# Autodesk Inventor assembly: Rack and Pinion Gearbox Assembly
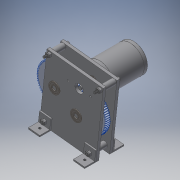
[picture p0: Inventor's stored thumbnail of the model, 180x180]
Saved by Autodesk Inventor 2018 (Build 220112000, 112)
## iProperties
Created: 2019-01-29
Part Number: Rack and Pinion Gearbox Assembly
Document SubType Name: Assembly
Designer: maste
Author: maste
## Documents named in this file (14)
- C:\Users\maste\OneDrive\Documents\GitHub\2019CAD\Drivebase but Calvin is a mad man\Rack and Pinion Gearbox Assembly.iam
- C:\Users\maste\OneDrive\Documents\GitHub\2019CAD\Drivebase but Calvin is a mad man\Rack and Pinion Gearbox Plate.ipt
- C:\Users\maste\OneDrive\Documents\GitHub\2019CAD\Drivebase but Calvin is a mad man\12t_Steel_Spur_Gear_20_DP_CIM_Motor_217-3099.ipt
- C:\Users\maste\OneDrive\Documents\GitHub\2019CAD\Drivebase but Calvin is a mad man\14t_Steel_Spur_Gear_20_DP_3_8_Hex_Bore_217-3100.step.ipt
- C:\Users\maste\OneDrive\Documents\GitHub\2019CAD\Drivebase but Calvin is a mad man\72t_Aluminum_Spur_Gear_20_DP_1_2_Hex_Bore_217-3576.ipt
- C:\Users\maste\OneDrive\Documents\GitHub\2019CAD\Drivebase but Calvin is a mad man\am-3832 375H to 500H Adapter.ipt
- C:\Users\maste\OneDrive\Documents\GitHub\2019CAD\Drivebase but Calvin is a mad man\Mini_CIM_Motor_217-3371.ipt
- C:\Users\maste\OneDrive\Documents\GitHub\2019CAD\Drivebase but Calvin is a mad man\10_25mm_3_8_ThunderHex_ID_x_0_875_OD_x_0_280_WD_Flanged_Bearing_217-5829 (1).ipt
- C:\Users\maste\OneDrive\Documents\GitHub\2019CAD\Drivebase but Calvin is a mad man\92196A272_18-8 STAINLESS STEEL SOCKET HEAD CAP SCREW.ipt
- C:\Users\maste\OneDrive\Documents\GitHub\2019CAD\Drivebase but Calvin is a mad man\Not Tiberculosis TB Hex Shaft.ipt
- C:\Users\maste\OneDrive\Documents\GitHub\2019CAD\Drivebase but Calvin is a mad man\I'm not awake enough to be making churros.ipt
- C:\Users\maste\OneDrive\Documents\GitHub\2019CAD\Drivebase but Calvin is a mad man\L-Bracket L.ipt
- C:\Users\maste\OneDrive\Documents\GitHub\2019CAD\Drivebase but Calvin is a mad man\92196A253_18-8 STAINLESS STEEL SOCKET HEAD CAP SCREW.ipt
- C:\Users\maste\OneDrive\Documents\GitHub\2019CAD\Drivebase but Calvin is a mad man\91831A011_TYPE 18-8 STAINLESS STL NYLON-INSERT LOCKNUT.ipt
## Components (33 placed, 13 different names)
1. Rack and Pinion Gearbox Plate:1 — Mate:1, Mate:2, Mate:3, Mate:6, Mate:7, Mate:8, Mate:9, Mate:10, Mate:11, Mate:12, Mate:13, Mate:20, Flush:3, Flush:4, Flush:8, Mate:48, Mate:49, Flush:9, Mate:50, Mate:51, Mate:52, Mate:53, Mate:56, Mate:57
2. Rack and Pinion Gearbox Plate:2 — Mate:24, Mate:25, Mate:26, Mate:27, Flush:3, Flush:4, Mate:36, Mate:37, Mate:38, Mate:39, Mate:40, Mate:41, Mate:42, Mate:43, Mate:44, Mate:45, Flush:6, Mate:46, Mate:47, Flush:7, Mate:60, Mate:61
3. 12t_Steel_Spur_Gear_20_DP_CIM_Motor_217-3099:1 — Mate:4, Mate:5, Flush:1
4. 14t_Steel_Spur_Gear_20_DP_3_8_Hex_Bore_217-3100.step:1 — Mate:21, Mate:22, Mate:23
5. 72t_Aluminum_Spur_Gear_20_DP_1_2_Hex_Bore_217-3576:1 — Mate:14, Mate:15, Flush:2, Mate:20, Mate:23, Mate:34
6. 72t_Aluminum_Spur_Gear_20_DP_1_2_Hex_Bore_217-3576:2 — Mate:30, Mate:31, Flush:5, Mate:34, Mate:35
7. am-3832 375H to 500H Adapter:1 — Mate:14, Mate:15, Flush:2, Mate:18, Mate:19
8. am-3832 375H to 500H Adapter:2 — Mate:30, Mate:31, Flush:5, Mate:32, Mate:33
9. Mini_CIM_Motor_217-3371:1 — Mate:1, Mate:2, Mate:3, Mate:4, Mate:5, Flush:1
10. 10_25mm_3_8_ThunderHex_ID_x_0_875_OD_x_0_280_WD_Flanged_Bearing_217-5829 (1):1 — Mate:24, Mate:25, Mate:35
11. 10_25mm_3_8_ThunderHex_ID_x_0_875_OD_x_0_280_WD_Flanged_Bearing_217-5829 (1):2 — Mate:26, Mate:27
12. 10_25mm_3_8_ThunderHex_ID_x_0_875_OD_x_0_280_WD_Flanged_Bearing_217-5829 (1):3 — Mate:8, Mate:9, Mate:28, Mate:29
13. 10_25mm_3_8_ThunderHex_ID_x_0_875_OD_x_0_280_WD_Flanged_Bearing_217-5829 (1):4 — Mate:6, Mate:7, Mate:16, Mate:17
14. 92196A272_18-8 STAINLESS STEEL SOCKET HEAD CAP SCREW:1 — Mate:10, Mate:13
15. 92196A272_18-8 STAINLESS STEEL SOCKET HEAD CAP SCREW:2 — Mate:11, Mate:12
16. Not Tiberculosis TB Hex Shaft:1 — Mate:16, Mate:17, Mate:18, Mate:19, Mate:21, Mate:22
17. Not Tiberculosis TB Hex Shaft:2 — Mate:28, Mate:29, Mate:32, Mate:33
18. I'm not awake enough to be making churros:1 — Mate:36, Mate:42
19. I'm not awake enough to be making churros:2 — Mate:38, Mate:43
20. I'm not awake enough to be making churros:3 — Mate:39, Mate:40
21. I'm not awake enough to be making churros:4 — Mate:37, Mate:41
22. L-Bracket L:1 — Flush:9, Mate:50, Mate:51, Mate:55, Mate:58
23. L-Bracket L:2 — Flush:8, Mate:48, Mate:49, Mate:54, Mate:59
24. L-Bracket L:3 — Mate:44, Mate:45, Flush:6, Mate:63
25. L-Bracket L:4 — Mate:46, Mate:47, Flush:7, Mate:62
26. 92196A253_18-8 STAINLESS STEEL SOCKET HEAD CAP SCREW:1 — Mate:54, Mate:59, Mate:65
27. 92196A253_18-8 STAINLESS STEEL SOCKET HEAD CAP SCREW:2 — Mate:55, Mate:58, Mate:64
28. 92196A253_18-8 STAINLESS STEEL SOCKET HEAD CAP SCREW:3 — Mate:52, Mate:56, Mate:67
29. 92196A253_18-8 STAINLESS STEEL SOCKET HEAD CAP SCREW:4 — Mate:53, Mate:57, Mate:66
30. 91831A011_TYPE 18-8 STAINLESS STL NYLON-INSERT LOCKNUT:1 — Mate:62, Mate:64
31. 91831A011_TYPE 18-8 STAINLESS STL NYLON-INSERT LOCKNUT:2 — Mate:63, Mate:65
32. 91831A011_TYPE 18-8 STAINLESS STL NYLON-INSERT LOCKNUT:3 — Mate:60, Mate:67
33. 91831A011_TYPE 18-8 STAINLESS STL NYLON-INSERT LOCKNUT:4 — Mate:61, Mate:66
## Relationships (76: Mate 67, Flush 9)
- Mate:1: Rack and Pinion Gearbox Plate:1 ↔ Mini_CIM_Motor_217-3371:1
- Mate:2: Rack and Pinion Gearbox Plate:1 ↔ Mini_CIM_Motor_217-3371:1
- Mate:3: Rack and Pinion Gearbox Plate:1 ↔ Mini_CIM_Motor_217-3371:1
- Mate:4: 12t_Steel_Spur_Gear_20_DP_CIM_Motor_217-3099:1 ↔ Mini_CIM_Motor_217-3371:1
- Mate:5: 12t_Steel_Spur_Gear_20_DP_CIM_Motor_217-3099:1 ↔ Mini_CIM_Motor_217-3371:1
- Flush:1: 12t_Steel_Spur_Gear_20_DP_CIM_Motor_217-3099:1 ↔ Mini_CIM_Motor_217-3371:1
- Mate:6: Rack and Pinion Gearbox Plate:1 ↔ 10_25mm_3_8_ThunderHex_ID_x_0_875_OD_x_0_280_WD_Flanged_Bearing_217-5829 (1):4
- Mate:7: Rack and Pinion Gearbox Plate:1 ↔ 10_25mm_3_8_ThunderHex_ID_x_0_875_OD_x_0_280_WD_Flanged_Bearing_217-5829 (1):4
- Mate:8: Rack and Pinion Gearbox Plate:1 ↔ 10_25mm_3_8_ThunderHex_ID_x_0_875_OD_x_0_280_WD_Flanged_Bearing_217-5829 (1):3
- Mate:9: Rack and Pinion Gearbox Plate:1 ↔ 10_25mm_3_8_ThunderHex_ID_x_0_875_OD_x_0_280_WD_Flanged_Bearing_217-5829 (1):3
- Mate:10: Rack and Pinion Gearbox Plate:1 ↔ 92196A272_18-8 STAINLESS STEEL SOCKET HEAD CAP SCREW:1
- Mate:11: Rack and Pinion Gearbox Plate:1 ↔ 92196A272_18-8 STAINLESS STEEL SOCKET HEAD CAP SCREW:2
- Mate:12: Rack and Pinion Gearbox Plate:1 ↔ 92196A272_18-8 STAINLESS STEEL SOCKET HEAD CAP SCREW:2
- Mate:13: Rack and Pinion Gearbox Plate:1 ↔ 92196A272_18-8 STAINLESS STEEL SOCKET HEAD CAP SCREW:1
- Mate:14: 72t_Aluminum_Spur_Gear_20_DP_1_2_Hex_Bore_217-3576:1 ↔ am-3832 375H to 500H Adapter:1
- Mate:15: 72t_Aluminum_Spur_Gear_20_DP_1_2_Hex_Bore_217-3576:1 ↔ am-3832 375H to 500H Adapter:1
- Flush:2: 72t_Aluminum_Spur_Gear_20_DP_1_2_Hex_Bore_217-3576:1 ↔ am-3832 375H to 500H Adapter:1
- Mate:16: 10_25mm_3_8_ThunderHex_ID_x_0_875_OD_x_0_280_WD_Flanged_Bearing_217-5829 (1):4 ↔ Not Tiberculosis TB Hex Shaft:1
- Mate:17: 10_25mm_3_8_ThunderHex_ID_x_0_875_OD_x_0_280_WD_Flanged_Bearing_217-5829 (1):4 ↔ Not Tiberculosis TB Hex Shaft:1
- Mate:18: am-3832 375H to 500H Adapter:1 ↔ Not Tiberculosis TB Hex Shaft:1
- Mate:19: am-3832 375H to 500H Adapter:1 ↔ Not Tiberculosis TB Hex Shaft:1
- Mate:20: Rack and Pinion Gearbox Plate:1 ↔ 72t_Aluminum_Spur_Gear_20_DP_1_2_Hex_Bore_217-3576:1
- Mate:21: 14t_Steel_Spur_Gear_20_DP_3_8_Hex_Bore_217-3100.step:1 ↔ Not Tiberculosis TB Hex Shaft:1
- Mate:22: 14t_Steel_Spur_Gear_20_DP_3_8_Hex_Bore_217-3100.step:1 ↔ Not Tiberculosis TB Hex Shaft:1
- Mate:23: 14t_Steel_Spur_Gear_20_DP_3_8_Hex_Bore_217-3100.step:1 ↔ 72t_Aluminum_Spur_Gear_20_DP_1_2_Hex_Bore_217-3576:1
- Mate:24: Rack and Pinion Gearbox Plate:2 ↔ 10_25mm_3_8_ThunderHex_ID_x_0_875_OD_x_0_280_WD_Flanged_Bearing_217-5829 (1):1
- Mate:25: Rack and Pinion Gearbox Plate:2 ↔ 10_25mm_3_8_ThunderHex_ID_x_0_875_OD_x_0_280_WD_Flanged_Bearing_217-5829 (1):1
- Mate:26: Rack and Pinion Gearbox Plate:2 ↔ 10_25mm_3_8_ThunderHex_ID_x_0_875_OD_x_0_280_WD_Flanged_Bearing_217-5829 (1):2
- Mate:27: Rack and Pinion Gearbox Plate:2 ↔ 10_25mm_3_8_ThunderHex_ID_x_0_875_OD_x_0_280_WD_Flanged_Bearing_217-5829 (1):2
- Flush:3: Rack and Pinion Gearbox Plate:1 ↔ Rack and Pinion Gearbox Plate:2
- Flush:4: Rack and Pinion Gearbox Plate:1 ↔ Rack and Pinion Gearbox Plate:2
- Mate:28: 10_25mm_3_8_ThunderHex_ID_x_0_875_OD_x_0_280_WD_Flanged_Bearing_217-5829 (1):3 ↔ Not Tiberculosis TB Hex Shaft:2
- Mate:29: 10_25mm_3_8_ThunderHex_ID_x_0_875_OD_x_0_280_WD_Flanged_Bearing_217-5829 (1):3 ↔ Not Tiberculosis TB Hex Shaft:2
- Mate:30: 72t_Aluminum_Spur_Gear_20_DP_1_2_Hex_Bore_217-3576:2 ↔ am-3832 375H to 500H Adapter:2
- Mate:31: 72t_Aluminum_Spur_Gear_20_DP_1_2_Hex_Bore_217-3576:2 ↔ am-3832 375H to 500H Adapter:2
- Flush:5: 72t_Aluminum_Spur_Gear_20_DP_1_2_Hex_Bore_217-3576:2 ↔ am-3832 375H to 500H Adapter:2
- Mate:32: am-3832 375H to 500H Adapter:2 ↔ Not Tiberculosis TB Hex Shaft:2
- Mate:33: am-3832 375H to 500H Adapter:2 ↔ Not Tiberculosis TB Hex Shaft:2
- Mate:34: 72t_Aluminum_Spur_Gear_20_DP_1_2_Hex_Bore_217-3576:1 ↔ 72t_Aluminum_Spur_Gear_20_DP_1_2_Hex_Bore_217-3576:2
- Mate:35: 72t_Aluminum_Spur_Gear_20_DP_1_2_Hex_Bore_217-3576:2 ↔ 10_25mm_3_8_ThunderHex_ID_x_0_875_OD_x_0_280_WD_Flanged_Bearing_217-5829 (1):1
- Mate:36: Rack and Pinion Gearbox Plate:2 ↔ I'm not awake enough to be making churros:1
- Mate:37: Rack and Pinion Gearbox Plate:2 ↔ I'm not awake enough to be making churros:4
- Mate:38: Rack and Pinion Gearbox Plate:2 ↔ I'm not awake enough to be making churros:2
- Mate:39: Rack and Pinion Gearbox Plate:2 ↔ I'm not awake enough to be making churros:3
- Mate:40: Rack and Pinion Gearbox Plate:2 ↔ I'm not awake enough to be making churros:3
- Mate:41: Rack and Pinion Gearbox Plate:2 ↔ I'm not awake enough to be making churros:4
- Mate:42: Rack and Pinion Gearbox Plate:2 ↔ I'm not awake enough to be making churros:1
- Mate:43: Rack and Pinion Gearbox Plate:2 ↔ I'm not awake enough to be making churros:2
- Mate:44: Rack and Pinion Gearbox Plate:2 ↔ L-Bracket L:3
- Mate:45: Rack and Pinion Gearbox Plate:2 ↔ L-Bracket L:3
- Flush:6: Rack and Pinion Gearbox Plate:2 ↔ L-Bracket L:3
- Mate:46: Rack and Pinion Gearbox Plate:2 ↔ L-Bracket L:4
- Mate:47: Rack and Pinion Gearbox Plate:2 ↔ L-Bracket L:4
- Flush:7: Rack and Pinion Gearbox Plate:2 ↔ L-Bracket L:4
- Flush:8: Rack and Pinion Gearbox Plate:1 ↔ L-Bracket L:2
- Mate:48: Rack and Pinion Gearbox Plate:1 ↔ L-Bracket L:2
- Mate:49: Rack and Pinion Gearbox Plate:1 ↔ L-Bracket L:2
- Flush:9: Rack and Pinion Gearbox Plate:1 ↔ L-Bracket L:1
- Mate:50: Rack and Pinion Gearbox Plate:1 ↔ L-Bracket L:1
- Mate:51: Rack and Pinion Gearbox Plate:1 ↔ L-Bracket L:1
- Mate:52: Rack and Pinion Gearbox Plate:1 ↔ 92196A253_18-8 STAINLESS STEEL SOCKET HEAD CAP SCREW:3
- Mate:53: Rack and Pinion Gearbox Plate:1 ↔ 92196A253_18-8 STAINLESS STEEL SOCKET HEAD CAP SCREW:4
- Mate:54: L-Bracket L:2 ↔ 92196A253_18-8 STAINLESS STEEL SOCKET HEAD CAP SCREW:1
- Mate:55: L-Bracket L:1 ↔ 92196A253_18-8 STAINLESS STEEL SOCKET HEAD CAP SCREW:2
- Mate:56: Rack and Pinion Gearbox Plate:1 ↔ 92196A253_18-8 STAINLESS STEEL SOCKET HEAD CAP SCREW:3
- Mate:57: Rack and Pinion Gearbox Plate:1 ↔ 92196A253_18-8 STAINLESS STEEL SOCKET HEAD CAP SCREW:4
- Mate:58: L-Bracket L:1 ↔ 92196A253_18-8 STAINLESS STEEL SOCKET HEAD CAP SCREW:2
- Mate:59: L-Bracket L:2 ↔ 92196A253_18-8 STAINLESS STEEL SOCKET HEAD CAP SCREW:1
- Mate:60: Rack and Pinion Gearbox Plate:2 ↔ 91831A011_TYPE 18-8 STAINLESS STL NYLON-INSERT LOCKNUT:3
- Mate:61: Rack and Pinion Gearbox Plate:2 ↔ 91831A011_TYPE 18-8 STAINLESS STL NYLON-INSERT LOCKNUT:4
- Mate:62: L-Bracket L:4 ↔ 91831A011_TYPE 18-8 STAINLESS STL NYLON-INSERT LOCKNUT:1
- Mate:63: L-Bracket L:3 ↔ 91831A011_TYPE 18-8 STAINLESS STL NYLON-INSERT LOCKNUT:2
- Mate:64: 92196A253_18-8 STAINLESS STEEL SOCKET HEAD CAP SCREW:2 ↔ 91831A011_TYPE 18-8 STAINLESS STL NYLON-INSERT LOCKNUT:1
- Mate:65: 92196A253_18-8 STAINLESS STEEL SOCKET HEAD CAP SCREW:1 ↔ 91831A011_TYPE 18-8 STAINLESS STL NYLON-INSERT LOCKNUT:2
- Mate:66: 92196A253_18-8 STAINLESS STEEL SOCKET HEAD CAP SCREW:4 ↔ 91831A011_TYPE 18-8 STAINLESS STL NYLON-INSERT LOCKNUT:4
- Mate:67: 92196A253_18-8 STAINLESS STEEL SOCKET HEAD CAP SCREW:3 ↔ 91831A011_TYPE 18-8 STAINLESS STL NYLON-INSERT LOCKNUT:3
